# Autodesk Inventor assembly: Grua Maya.ipt
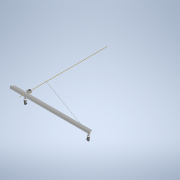
[picture p0: Inventor's stored thumbnail of the model, 180x180]
Saved by Autodesk Inventor 2020 (Build 240168000, 168)
## iProperties
Created: 2019-10-05
Part Number: Grua Maya.ipt
Document SubType Name: Assembly
Designer: dasa1
Author: dasa1
## Documents named in this file (4)
- C:\Users\dasa1\OneDrive\Documents\Inventor\Virtualización Maya\Grua Maya.ipt.iam
- C:\Users\dasa1\OneDrive\Documents\Inventor\Virtualización Maya\Grua Maya.ipt
- C:\Users\dasa1\OneDrive\Documents\Inventor\Virtualización Maya\motor.ipt
- C:\Users\dasa1\OneDrive\Documents\Inventor\Virtualización Maya\140w-servo-integrated-motor-1.snapshot.4\LG100 089.ipt
## Components (4 placed, 3 different names)
1. Grua Maya:1 — Ángulo:1, Coincidencia:1, Nivelación:2, Nivelación:3, Coincidencia:2, Coincidencia:3, Coincidencia:4, Ángulo:2, Nivelación:4, Coincidencia:5, Nivelación:5
2. motor:1 — Ángulo:1, Coincidencia:1, Nivelación:2, Nivelación:3
3. LG100 089:1 — Coincidencia:2, Coincidencia:4, Coincidencia:5
4. LG100 089:2 — Coincidencia:3, Ángulo:2, Nivelación:4, Nivelación:5
## Relationships (11: Mate 5, Flush 4, Angle 2)
- Ángulo:1 [Angle] (0 deg): Grua Maya:1 ↔ motor:1
- Coincidencia:1 [Mate]: Grua Maya:1 ↔ motor:1
- Nivelación:2 [Flush]: Grua Maya:1 ↔ motor:1
- Nivelación:3 [Flush] (-65 mm): Grua Maya:1 ↔ motor:1
- Coincidencia:2 [Mate]: Grua Maya:1 ↔ LG100 089:1
- Coincidencia:3 [Mate]: Grua Maya:1 ↔ LG100 089:2
- Coincidencia:4 [Mate] (10 mm): Grua Maya:1 ↔ LG100 089:1
- Ángulo:2 [Angle] (0 deg): Grua Maya:1 ↔ LG100 089:2
- Nivelación:4 [Flush]: Grua Maya:1 ↔ LG100 089:2
- Coincidencia:5 [Mate] (-12 mm): Grua Maya:1 ↔ LG100 089:1
- Nivelación:5 [Flush]: Grua Maya:1 ↔ LG100 089:2
